# Autodesk Inventor assembly: NRF24L01L+Antenna 90
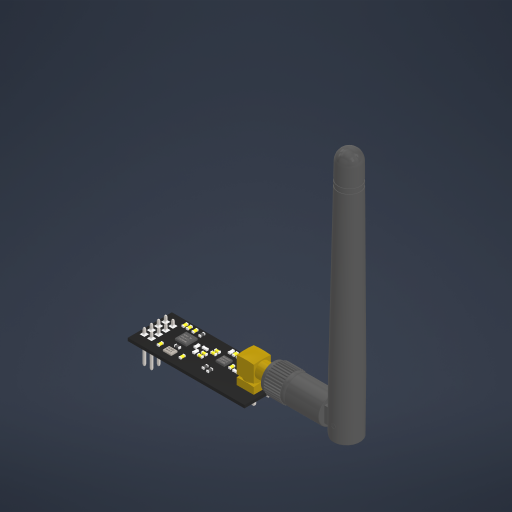
[picture p0: Inventor's stored thumbnail of the model, 512x512]
Saved by Autodesk Inventor 2024 (Build 280153000, 153)
## iProperties
Created: 2021-06-04
Part Number: NRF24L01L+Antenna 90
Description: STEP AP214
Document SubType Name: Assembly
Designer: Vincent Larson
Sending System: SolidWorks 2016
Preprocessor: SwSTEP 2.0
Title: NRF24L01L+Antenna.STEP
Revision Number: ANY
## Documents named in this file (3)
- C:\Users\Vincent Larson\Downloads\Digital Ship Challenge\Digital Ship Challenge Robot\NRF24L01L+Antenna\NRF24L01L+Antenna 90.iam
- C:\Users\Vincent Larson\Downloads\Digital Ship Challenge\Digital Ship Challenge Robot\NRF24L01L+Antenna\NRF24L01L.ipt
- C:\Users\Vincent Larson\Downloads\Digital Ship Challenge\Digital Ship Challenge Robot\NRF24L01L+Antenna\Antenna assy_90.iam
## Components (2 placed, 2 different names)
1. NRF24L01L_1 — Mate:1
2. Antenna assy_90:1 [sub-assembly] — Mate:1
## Relationships (1: Mate 1)
- Mate:1: NRF24L01L_1 ↔ Antenna assy_90:1
